# Autodesk Inventor assembly: robot_simu
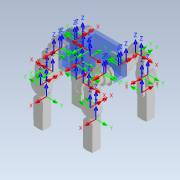
[picture p0: Inventor's stored thumbnail of the model, 180x180]
Saved by Autodesk Inventor 2020 (Build 240168000, 168)
## iProperties
Created: 2021-01-12
Part Number: robot_simu
Document SubType Name: Assembly
Designer: DELL
Author: DELL
## Documents named in this file (13)
- F:\SoftRobot2.0\FlexipodHardware2.0\FlexipodHardware\Flexipod2.0\Cadquery_module\v3.0\robot_simu.iam
- F:\SoftRobot2.0\FlexipodHardware2.0\FlexipodHardware\Flexipod2.0\Cadquery_module\v3.0\body.ipt
- F:\SoftRobot2.0\FlexipodHardware2.0\FlexipodHardware\Flexipod2.0\Cadquery_module\v3.0\body_motor_fix_board_left.ipt
- F:\SoftRobot2.0\FlexipodHardware2.0\FlexipodHardware\Flexipod2.0\Cadquery_module\v3.0\body_motor_fix_board_right.ipt
- F:\SoftRobot2.0\FlexipodHardware2.0\FlexipodHardware\Flexipod2.0\Cadquery_module\v3.0\motor.ipt
- F:\SoftRobot2.0\FlexipodHardware2.0\FlexipodHardware\Flexipod2.0\Cadquery_module\v3.0\hip_front_left.ipt
- F:\SoftRobot2.0\FlexipodHardware2.0\FlexipodHardware\Flexipod2.0\Cadquery_module\v3.0\hip_front_right.ipt
- F:\SoftRobot2.0\FlexipodHardware2.0\FlexipodHardware\Flexipod2.0\Cadquery_module\v3.0\left_thigh.ipt
- F:\SoftRobot2.0\FlexipodHardware2.0\FlexipodHardware\Flexipod2.0\Cadquery_module\v3.0\right_thigh.ipt
- F:\SoftRobot2.0\FlexipodHardware2.0\FlexipodHardware\Flexipod2.0\Cadquery_module\v3.0\shank_board.ipt
- F:\SoftRobot2.0\FlexipodHardware2.0\FlexipodHardware\Flexipod2.0\Cadquery_module\v3.0\shank.ipt
- F:\SoftRobot2.0\FlexipodHardware2.0\FlexipodHardware\Flexipod2.0\Cadquery_module\v3.0\hip_back_left.ipt
- F:\SoftRobot2.0\FlexipodHardware2.0\FlexipodHardware\Flexipod2.0\Cadquery_module\v3.0\hip_back_right.ipt
## Components (33 placed, 12 different names)
1. body:1 — Mate:1, Flush:1, Flush:2, Flush:3, Flush:4, Flush:5, Mate:2, Flush:6, Flush:7, Mate:3, Flush:8, Flush:9, Mate:4, Flush:10, Flush:11, Mate:5, Angle:1, Mate:7, Angle:2, Mate:9, Angle:3, Mate:10, Angle:4, Angle:5, Angle:6, Angle:8, Angle:9, Angle:10, Angle:17, Angle:18, Angle:19, Angle:20, Angle:21, Angle:22
2. body_motor_fix_board_left:1 — Mate:1, Flush:1, Flush:2, Mate:6
3. body_motor_fix_board_left:2 — Mate:3, Flush:8, Flush:9, Mate:18
4. body_motor_fix_board_right:1 — Mate:4, Flush:10, Flush:11, Mate:11
5. body_motor_fix_board_right:2 — Mate:2, Flush:6, Flush:7, Mate:8
6. motor:1 — Mate:5, Mate:6, Angle:1, Mate:14, Mate:15
7. motor:2 — Mate:7, Mate:8, Angle:2, Mate:12, Mate:13
8. motor:3 — Mate:9, Angle:3, Mate:18, Mate:39, Mate:40
9. motor:4 — Mate:10, Mate:11, Angle:4, Mate:37, Mate:38
10. hip_front_left:1 — Mate:14, Mate:15, Angle:6, Mate:16, Mate:17, Angle:7
11. hip_front_right:1 — Mate:12, Mate:13, Angle:5, Mate:19, Mate:20
12. motor:5 — Mate:16, Mate:17, Angle:7, Mate:21, Mate:22
13. motor:6 — Mate:19, Mate:20, Angle:8, Mate:23, Mate:24
14. left_thigh:1 — Mate:21, Mate:22, Angle:9, Mate:27, Mate:28, Angle:12, Angle:13
15. right_thigh:1 — Mate:23, Mate:24, Angle:10, Mate:25, Mate:26, Angle:11, Angle:14
16. motor:7 — Mate:25, Mate:26, Angle:11, Mate:31, Mate:32
17. motor:8 — Mate:27, Mate:28, Angle:12, Mate:29, Mate:30
18. shank_board:1 — Mate:31, Mate:32, Angle:14, Mate:33, Mate:34, Angle:16
19. shank_board:2 — Mate:29, Mate:30, Angle:13, Mate:35, Mate:36, Angle:15
20. shank:1 — Mate:35, Mate:36, Angle:15
21. shank:2 — Mate:33, Mate:34, Angle:16
22. hip_back_left:1 — Mate:39, Mate:40, Angle:18, Mate:43, Mate:44
23. hip_back_right:1 — Mate:37, Mate:38, Angle:17, Mate:41, Mate:42
24. motor:9 — Mate:41, Mate:42, Angle:19, Mate:45, Mate:46
25. motor:10 — Mate:43, Mate:44, Angle:20, Mate:47, Mate:48
26. left_thigh:2 — Mate:47, Mate:48, Angle:22, Mate:51, Mate:52, Angle:24, Angle:26, Angle:28
27. right_thigh:2 — Mate:45, Mate:46, Angle:21, Mate:49, Mate:50, Angle:23, Angle:25, Angle:27
28. motor:11 — Mate:49, Mate:50, Angle:23, Mate:53, Mate:55
29. motor:12 — Mate:51, Mate:52, Angle:24, Mate:54, Mate:56
30. shank_board:3 — Mate:54, Mate:56, Angle:26, Mate:59, Mate:60
31. shank_board:4 — Mate:53, Mate:55, Angle:25, Mate:57, Mate:58
32. shank:3 — Mate:57, Mate:58, Angle:27
33. shank:4 — Mate:59, Mate:60, Angle:28
## Relationships (99: Mate 60, Angle 28, Flush 11)
- Mate:1: body:1 ↔ body_motor_fix_board_left:1
- Flush:1: body:1 ↔ body_motor_fix_board_left:1
- Flush:2: body:1 ↔ body_motor_fix_board_left:1
- Flush:3: body:1
- Flush:4: body:1
- Flush:5: body:1
- Mate:2: body:1 ↔ body_motor_fix_board_right:2
- Flush:6: body:1 ↔ body_motor_fix_board_right:2
- Flush:7: body:1 ↔ body_motor_fix_board_right:2
- Mate:3: body:1 ↔ body_motor_fix_board_left:2
- Flush:8: body:1 ↔ body_motor_fix_board_left:2
- Flush:9: body:1 ↔ body_motor_fix_board_left:2
- Mate:4: body:1 ↔ body_motor_fix_board_right:1
- Flush:10: body:1 ↔ body_motor_fix_board_right:1
- Flush:11: body:1 ↔ body_motor_fix_board_right:1
- Mate:5: body:1 ↔ motor:1
- Mate:6: body_motor_fix_board_left:1 ↔ motor:1
- Angle:1 (180 deg): body:1 ↔ motor:1
- Mate:7: body:1 ↔ motor:2
- Mate:8: body_motor_fix_board_right:2 ↔ motor:2
- Angle:2 (0 deg): body:1 ↔ motor:2
- Mate:9: body:1 ↔ motor:3
- Angle:3 (180 deg): body:1 ↔ motor:3
- Mate:10: body:1 ↔ motor:4
- Mate:11: body_motor_fix_board_right:1 ↔ motor:4
- Angle:4 (0 deg): body:1 ↔ motor:4
- Mate:12: motor:2 ↔ hip_front_right:1
- Mate:13: motor:2 ↔ hip_front_right:1
- Angle:5 (0 deg): body:1 ↔ hip_front_right:1
- Mate:14: motor:1 ↔ hip_front_left:1
- Mate:15: motor:1 ↔ hip_front_left:1
- Angle:6 (0 deg): body:1 ↔ hip_front_left:1
- Mate:16: hip_front_left:1 ↔ motor:5
- Mate:17: hip_front_left:1 ↔ motor:5
- Angle:7 (0 deg): hip_front_left:1 ↔ motor:5
- Mate:18: body_motor_fix_board_left:2 ↔ motor:3
- Mate:19: hip_front_right:1 ↔ motor:6
- Mate:20: hip_front_right:1 ↔ motor:6
- Angle:8 (180 deg): body:1 ↔ motor:6
- Mate:21: motor:5 ↔ left_thigh:1
- Mate:22: motor:5 ↔ left_thigh:1
- Angle:9 (0 deg): body:1 ↔ left_thigh:1
- Mate:23: motor:6 ↔ right_thigh:1
- Mate:24: motor:6 ↔ right_thigh:1
- Angle:10 (0 deg): body:1 ↔ right_thigh:1
- Mate:25: right_thigh:1 ↔ motor:7
- Mate:26: right_thigh:1 ↔ motor:7
- Angle:11 (180 deg): right_thigh:1 ↔ motor:7
- Mate:27: left_thigh:1 ↔ motor:8
- Mate:28: left_thigh:1 ↔ motor:8
- Angle:12 (0 deg): left_thigh:1 ↔ motor:8
- Mate:29: motor:8 ↔ shank_board:2
- Mate:30: motor:8 ↔ shank_board:2
- Angle:13 (0 deg): left_thigh:1 ↔ shank_board:2
- Mate:31: motor:7 ↔ shank_board:1
- Mate:32: motor:7 ↔ shank_board:1
- Angle:14 (0 deg): right_thigh:1 ↔ shank_board:1
- Mate:33: shank_board:1 ↔ shank:2
- Mate:34: shank_board:1 ↔ shank:2
- Mate:35: shank_board:2 ↔ shank:1
- Mate:36: shank_board:2 ↔ shank:1
- Angle:15 (180 deg): shank_board:2 ↔ shank:1
- Angle:16 (0 deg): shank_board:1 ↔ shank:2
- Mate:37: motor:4 ↔ hip_back_right:1
- Mate:38: motor:4 ↔ hip_back_right:1
- Angle:17 (0 deg): body:1 ↔ hip_back_right:1
- Mate:39: motor:3 ↔ hip_back_left:1
- Mate:40: motor:3 ↔ hip_back_left:1
- Angle:18 (0 deg): body:1 ↔ hip_back_left:1
- Mate:41: hip_back_right:1 ↔ motor:9
- Mate:42: hip_back_right:1 ↔ motor:9
- Mate:43: hip_back_left:1 ↔ motor:10
- Mate:44: hip_back_left:1 ↔ motor:10
- Angle:19 (180 deg): body:1 ↔ motor:9
- Angle:20 (0 deg): body:1 ↔ motor:10
- Mate:45: motor:9 ↔ right_thigh:2
- Mate:46: motor:9 ↔ right_thigh:2
- Mate:47: motor:10 ↔ left_thigh:2
- Mate:48: motor:10 ↔ left_thigh:2
- Angle:21 (0 deg): body:1 ↔ right_thigh:2
- Angle:22 (0 deg): body:1 ↔ left_thigh:2
- Mate:49: right_thigh:2 ↔ motor:11
- Mate:50: right_thigh:2 ↔ motor:11
- Mate:51: left_thigh:2 ↔ motor:12
- Mate:52: left_thigh:2 ↔ motor:12
- Angle:23 (180 deg): right_thigh:2 ↔ motor:11
- Angle:24 (0 deg): left_thigh:2 ↔ motor:12
- Mate:53: motor:11 ↔ shank_board:4
- Mate:54: motor:12 ↔ shank_board:3
- Mate:55: motor:11 ↔ shank_board:4
- Mate:56: motor:12 ↔ shank_board:3
- Angle:25 (0 deg): right_thigh:2 ↔ shank_board:4
- Angle:26 (0 deg): left_thigh:2 ↔ shank_board:3
- Mate:57: shank_board:4 ↔ shank:3
- Mate:58: shank_board:4 ↔ shank:3
- Mate:59: shank_board:3 ↔ shank:4
- Mate:60: shank_board:3 ↔ shank:4
- Angle:27 (0 deg): right_thigh:2 ↔ shank:3
- Angle:28 (180 deg): left_thigh:2 ↔ shank:4
